# Autodesk Inventor assembly: Mais uma montagem
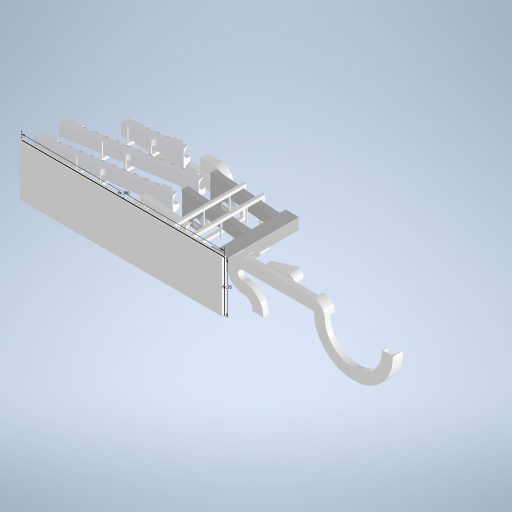
[picture p0: Inventor's stored thumbnail of the model, 512x512]
Saved by Autodesk Inventor 2024 (Build 280153000, 153)
## iProperties
Created: 2023-05-12
Part Number: Mais uma montagem
Document SubType Name: Assembly
Designer: jpjoa
Author: jpjoa
## Documents named in this file (15)
- G:\.shortcut-targets-by-id\1lOMf-Kp8UroJbDMtxyO7ak_I_KYCWiat\Faculdade\Trabalhos\Desenho e Print 3D\Marbles project\Montagem final.iam
- G:\.shortcut-targets-by-id\1lOMf-Kp8UroJbDMtxyO7ak_I_KYCWiat\Faculdade\Trabalhos\Desenho e Print 3D\Marbles project\Base.ipt
- G:\.shortcut-targets-by-id\1lOMf-Kp8UroJbDMtxyO7ak_I_KYCWiat\Faculdade\Trabalhos\Desenho e Print 3D\Marbles project\Box de reinício.ipt
- G:\.shortcut-targets-by-id\1lOMf-Kp8UroJbDMtxyO7ak_I_KYCWiat\Faculdade\Trabalhos\Desenho e Print 3D\Marbles project\Conector superior para giro.ipt
- G:\.shortcut-targets-by-id\1lOMf-Kp8UroJbDMtxyO7ak_I_KYCWiat\Faculdade\Trabalhos\Desenho e Print 3D\Marbles project\Parafuso.ipt
- G:\.shortcut-targets-by-id\1lOMf-Kp8UroJbDMtxyO7ak_I_KYCWiat\Faculdade\Trabalhos\Desenho e Print 3D\Marbles project\Receptor pequeno.ipt
- G:\.shortcut-targets-by-id\1lOMf-Kp8UroJbDMtxyO7ak_I_KYCWiat\Faculdade\Trabalhos\Desenho e Print 3D\Marbles project\Sustentação Trilhos fixos.ipt
- G:\.shortcut-targets-by-id\1lOMf-Kp8UroJbDMtxyO7ak_I_KYCWiat\Faculdade\Trabalhos\Desenho e Print 3D\Marbles project\Sustentação Trilhos.ipt
- G:\.shortcut-targets-by-id\1lOMf-Kp8UroJbDMtxyO7ak_I_KYCWiat\Faculdade\Trabalhos\Desenho e Print 3D\Marbles project\Troca de sentido.ipt
- G:\.shortcut-targets-by-id\1lOMf-Kp8UroJbDMtxyO7ak_I_KYCWiat\Faculdade\Trabalhos\Desenho e Print 3D\Marbles project\Libera todas.ipt
- G:\.shortcut-targets-by-id\1lOMf-Kp8UroJbDMtxyO7ak_I_KYCWiat\Faculdade\Trabalhos\Desenho e Print 3D\Marbles project\Marbles - Peças novas\Pega uma e libera maior.ipt
- G:\.shortcut-targets-by-id\1lOMf-Kp8UroJbDMtxyO7ak_I_KYCWiat\Faculdade\Trabalhos\Desenho e Print 3D\Marbles project\Marbles - Peças novas\Pega uma e libera menor.ipt
- G:\.shortcut-targets-by-id\1lOMf-Kp8UroJbDMtxyO7ak_I_KYCWiat\Faculdade\Trabalhos\Desenho e Print 3D\Marbles project\Marbles - Peças novas\Trilho 60 min - 12 horas montado.iam
- G:\.shortcut-targets-by-id\1lOMf-Kp8UroJbDMtxyO7ak_I_KYCWiat\Faculdade\Trabalhos\Desenho e Print 3D\Marbles project\Marbles - Peças novas\Trilho 5 min montado.iam
- G:\.shortcut-targets-by-id\1lOMf-Kp8UroJbDMtxyO7ak_I_KYCWiat\Faculdade\Trabalhos\Desenho e Print 3D\Marbles project\Agrupar bolinhas novamente.ipt
## Components (27 placed, 14 different names)
1. Base:1 — Alinhado:2, Coincidente:1, Coincidente:3, Alinhado:14, Coincidente:12, Coincidente:13, Coincidente:14, Coincidente:16, Coincidente:32
2. Box de reinício:1 — Alinhado:2, Coincidente:1, Coincidente:4, Alinhado:21, Coincidente:19, Alinhado:23, Alinhado:26, Coincidente:26, Coincidente:27, Alinhado:27, Coincidente:28, Coincidente:29, Alinhado:28, Coincidente:30, Coincidente:31, Inserir:30
3. Conector superior para giro:1 — Inserir:4
4. Receptor pequeno:1 — Alinhado:19
5. Sustentação Trilhos fixos:1 — Coincidente:3, Coincidente:4, Alinhado:14, Alinhado:20, Rígida:1, Inserir:10, Inserir:11, Inserir:12, Inserir:13, Inserir:14, Coincidente:15, Alinhado:22
6. Sustentação Trilhos:1 — Coincidente:16, Inserir:18, Inserir:19, Inserir:20, Inserir:21, Inserir:22, Inserir:23, Coincidente:18, Coincidente:19
7. Troca de sentido:1 — Inserir:4
8. Receptor pequeno:2 — Alinhado:19
9. Parafuso:2 — Inserir:10
10. Parafuso:3 — Inserir:11
11. Parafuso:4 — Inserir:12
12. Parafuso:5 — Inserir:13
13. Parafuso:6 — Alinhado:20, Rígida:1
14. Parafuso:7 — Inserir:14
15. Parafuso:8 — Inserir:22
16. Parafuso:9 — Inserir:21, Inserir:29
17. Parafuso:10 — Inserir:18, Inserir:28
18. Parafuso:11 — Inserir:23
19. Parafuso:12 — Inserir:20, Inserir:27
20. Parafuso:13 — Inserir:19
21. Libera todas:1 — Alinhado:23, Alinhado:26, Coincidente:26, Coincidente:27
22. Pega uma e libera maior:1 — Alinhado:27, Coincidente:28, Coincidente:29
23. Pega uma e libera menor:1 — Alinhado:28, Coincidente:30, Coincidente:31
24. Trilho 60 min - 12 horas montado:1 [sub-assembly] — Inserir:27
25. Trilho 5 min montado:1 [sub-assembly] — Inserir:28
26. Trilho 60 min - 12 horas montado:2 [sub-assembly] — Inserir:29
27. Agrupar bolinhas novamente:1 — Coincidente:32, Inserir:30
## Relationships (44: Mate 17, Insert 16, Flush 10, WeldJoint 1)
- Alinhado:2 [Flush]: Base:1 ↔ Box de reinício:1
- Coincidente:1 [Mate]: Base:1 ↔ Box de reinício:1
- Inserir:4: Conector superior para giro:1 ↔ Troca de sentido:1
- Coincidente:3 [Mate]: Base:1 ↔ Sustentação Trilhos fixos:1
- Coincidente:4 [Mate]: Box de reinício:1 ↔ Sustentação Trilhos fixos:1
- Alinhado:14 [Flush]: Base:1 ↔ Sustentação Trilhos fixos:1
- Alinhado:19 [Flush]: Receptor pequeno:1 ↔ Receptor pequeno:2
- Coincidente:12 [Mate]: Base:1
- Coincidente:13 [Mate]: Base:1
- Coincidente:14 [Mate]: Base:1
- Alinhado:20 [Flush]: Sustentação Trilhos fixos:1 ↔ Parafuso:6
- Rígida:1 [WeldJoint]: Sustentação Trilhos fixos:1 ↔ Parafuso:6
- Inserir:10: Sustentação Trilhos fixos:1 ↔ Parafuso:2
- Inserir:11: Sustentação Trilhos fixos:1 ↔ Parafuso:3
- Inserir:12: Sustentação Trilhos fixos:1 ↔ Parafuso:4
- Inserir:13: Sustentação Trilhos fixos:1 ↔ Parafuso:5
- Inserir:14: Sustentação Trilhos fixos:1 ↔ Parafuso:7
- Alinhado:21 [Flush] (73.935 mm): Box de reinício:1
- Coincidente:15 [Mate]: Sustentação Trilhos fixos:1
- Coincidente:16 [Mate]: Base:1 ↔ Sustentação Trilhos:1
- Inserir:18: Sustentação Trilhos:1 ↔ Parafuso:10
- Inserir:19: Sustentação Trilhos:1 ↔ Parafuso:13
- Inserir:20: Sustentação Trilhos:1 ↔ Parafuso:12
- Inserir:21: Sustentação Trilhos:1 ↔ Parafuso:9
- Inserir:22: Sustentação Trilhos:1 ↔ Parafuso:8
- Inserir:23: Sustentação Trilhos:1 ↔ Parafuso:11
- Alinhado:22 [Flush] (156.718 mm): Sustentação Trilhos fixos:1
- Coincidente:18 [Mate]: Sustentação Trilhos:1
- Coincidente:19 [Mate]: Box de reinício:1 ↔ Sustentação Trilhos:1
- Alinhado:23 [Flush]: Box de reinício:1 ↔ Libera todas:1
- Inserir:27: Parafuso:12 ↔ Trilho 60 min - 12 horas montado:1
- Inserir:28: Parafuso:10 ↔ Trilho 5 min montado:1
- Inserir:29: Parafuso:9 ↔ Trilho 60 min - 12 horas montado:2
- Alinhado:26 [Flush]: Box de reinício:1 ↔ Libera todas:1
- Coincidente:26 [Mate]: Box de reinício:1 ↔ Libera todas:1
- Coincidente:27 [Mate]: Box de reinício:1 ↔ Libera todas:1
- Alinhado:27 [Flush]: Box de reinício:1 ↔ Pega uma e libera maior:1
- Coincidente:28 [Mate]: Box de reinício:1 ↔ Pega uma e libera maior:1
- Coincidente:29 [Mate]: Box de reinício:1 ↔ Pega uma e libera maior:1
- Alinhado:28 [Flush]: Box de reinício:1 ↔ Pega uma e libera menor:1
- Coincidente:30 [Mate]: Box de reinício:1 ↔ Pega uma e libera menor:1
- Coincidente:31 [Mate]: Box de reinício:1 ↔ Pega uma e libera menor:1
- Coincidente:32 [Mate]: Base:1 ↔ Agrupar bolinhas novamente:1
- Inserir:30: Box de reinício:1 ↔ Agrupar bolinhas novamente:1
